# Autodesk Inventor assembly: trmometr
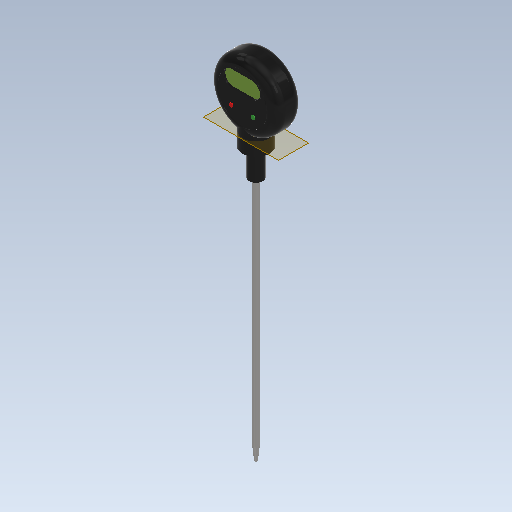
[picture p0: Inventor's stored thumbnail of the model, 512x512]
Saved by Autodesk Inventor 2021 (Build 250183000, 183)
## iProperties
Created: 2021-05-20
Part Number: trmometr
Document SubType Name: Assembly
Designer: Wojciech Wołczek
Author: Wojciech Wołczek
## Documents named in this file (3)
- D:\OneDrive\Documents\studia\I rok\labolatoria pracowni fizycznej\pracownia fizyczna 2021 xD\cw 25\trmometr.iam
- D:\OneDrive\Documents\studia\I rok\labolatoria pracowni fizycznej\pracownia fizyczna 2021 xD\cw 25\top temp.ipt
- D:\OneDrive\Documents\studia\I rok\labolatoria pracowni fizycznej\pracownia fizyczna 2021 xD\cw 25\bolec.ipt
## Components (2 placed, 2 different names)
1. top temp:1 — Równoległe:1
2. bolec:1 — Równoległe:1
## Relationships (1: Flush 1)
- Równoległe:1 [Flush]: top temp:1 ↔ bolec:1
